# Autodesk Inventor assembly: benchvice
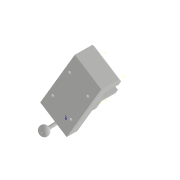
[picture p0: Inventor's stored thumbnail of the model, 180x180]
Saved by Autodesk Inventor 2020 (Build 240168000, 168)
## iProperties
Created: 2021-12-10
Part Number: benchvice
Document SubType Name: Assembly
Designer: NIKHIL VINOD
Author: NIKHIL VINOD
## Documents named in this file (9)
- C:\Users\NIKHIL VINOD\Desktop\benchvice.iam
- C:\Users\NIKHIL VINOD\Desktop\first.ipt
- C:\Users\NIKHIL VINOD\Desktop\second.ipt
- C:\Users\NIKHIL VINOD\Desktop\third.ipt
- C:\Users\NIKHIL VINOD\Desktop\eighth.ipt
- C:\Users\NIKHIL VINOD\Desktop\four.ipt
- C:\Users\NIKHIL VINOD\Desktop\seventh.ipt
- C:\Users\NIKHIL VINOD\Desktop\fifth.ipt
- C:\Users\NIKHIL VINOD\Desktop\sixth.ipt
## Components (9 placed, 8 different names)
1. first:1 — Mate:1, Mate:2, Mate:3, Mate:4, Mate:9, Mate:12, Mate:19, Mate:23
2. second:1 — Mate:5, Mate:6, Mate:7, Mate:8, Mate:9, Mate:10, Mate:11
3. third:1 — Mate:13, Mate:14, Mate:19, Mate:27, Mate:28
4. eighth:1 — Mate:11, Mate:12, Mate:15, Mate:16
5. fifth:1 — Mate:23, Mate:24
6. four:1 — Mate:24, Mate:25, Mate:26, Rotational:1
7. seventh:1 — Mate:25, Mate:26
8. seventh:2 — Rotational:1
9. sixth:1 — Mate:27, Mate:28
## Relationships (26: Mate 25, RevoluteJoint 1)
- Mate:1: first:1
- Mate:2: first:1
- Mate:3: first:1
- Mate:4: first:1
- Mate:5: second:1
- Mate:6: second:1
- Mate:7: second:1
- Mate:8: second:1
- Mate:9: first:1 ↔ second:1
- Mate:10: second:1
- Mate:11: second:1 ↔ eighth:1
- Mate:12: first:1 ↔ eighth:1
- Mate:13: third:1
- Mate:14: third:1
- Mate:15: eighth:1
- Mate:16: eighth:1
- Mate:17
- Mate:18
- Mate:19: first:1 ↔ third:1
- Mate:23: first:1 ↔ fifth:1
- Mate:24: fifth:1 ↔ four:1
- Mate:25: four:1 ↔ seventh:1
- Mate:26: four:1 ↔ seventh:1
- Rotational:1 [RevoluteJoint]: four:1 ↔ seventh:2
- Mate:27: third:1 ↔ sixth:1
- Mate:28: third:1 ↔ sixth:1
